# Autodesk Inventor assembly: SCLBRU5-35.0
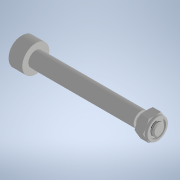
[picture p0: Inventor's stored thumbnail of the model, 180x180]
Saved by Autodesk Inventor 2021 (Build 250183000, 183)
## iProperties
Category: PARTsolutions
Company: MISUMI
Created: 2025-08-07
Part Number: SCLBRU5-35.0
Catalog Web Link: www.cadenas.de
Description: CLBR, CLBRH, PCLBR, PCLBRH, GCLBR, SCLBR, SCLBRH, GSCLBR, CLBRU, CLBRHU, PCLBRU, PCLBRHU, GCLBRU, SCLBRU, SCLBRHU, GSCLBRU-Hinge Pins - Lock Nut Type with Hexagon Socket Head
Vendor: MISUMI
Document SubType Name: Assembly
Designer: psAdmin
Manufacturer: MISUMI
Mass: 1.17278 g
Surface Area: 11.0588 cm^2
Volume: 1.17278 cm^3
Density: 1 g/cm^3
Title: SCLBRU5-35.0
Author: Cadenas PARTsolutions
Comments: Hinge Pins - Lock Nut Type with Hexagon Socket Head
PSOL_IDENT_0: {$CADENAS_DATA/23d-libs/misumi/metric/13_cantilever_shafts/clbr_asmtab.prj},343 {VTYP=3D},{STYP=ASST
PSOL_IDENT_1: AB},{NB=SCLBRU5-35.0},{LINA=SCLBRU5-35.0},{NN=CLBR, CLBRH, PCLBR, PCLBRH, GCLBR, SCLBR, SCLBRH, GSCL
PSOL_IDENT_2: BR, CLBRU, CLBRHU, PCLBRU, PCLBRHU, GCLBRU, SCLBRU, SCLBRHU, GSCLBRU},{DATE=21.04.2022 08:37:10},{GE
PSOL_IDENT_3: OMDATE=17.06.2021 12:28:52},{VERSION=},{LINEID=30},{WBVAR=MAT,HARD,ST,AC,L,ALT3,ALT2,MC,ALT1,FC,ALT4
PSOL_IDENT_4: },{WBNUMERIC=L,MC,FC}  {NB=SCLBRU5-35.0},{LINA=SCLBRU5-35.0},{KT=DUMMY},{PN=SCLBRU5-35.0},{TYPE=SCLB
PSOL_IDENT_5: RU},{MAT=SUS304},{HARD=1},{HARDALG= '1', '-' },{ST=},{STALG= '', '-' },{AC=UN},{ACALG= 'SN', 'Standa
PSOL_IDENT_6: rd Nuts', 'UN', 'U-Nuts' },{MATAC1=304 Stainless Steel (UNUTS)},{MATAC2=0},{STAC=0},{D=5},{L=35.0},{
PSOL_IDENT_7: L1=[10.0:100.0/0.1]},{LPN=35.0},{LPN1=35},{LPN2=0},{ALT3=},{A=9},{T=5},{ALT2=},{ALT2ALG= '' , 'Not a
PSOL_IDENT_8: pplicable' },{ALT2PN=},{MC=0},{MCALG=0},{M=M4},{M1=4},{M3D=4},{ALT1=},{ALT1ALG= '', 'w/o FC (Thread
PSOL_IDENT_9: Part Length)', '-FC', 'with FC (Thread Part Length)' },{ALT1PN=},{FC=0},{FCALG=0},{FCMIN1=4},{FCMAX1=
PSOL_IDENT_10: 5},{FCMIN2=7},{FCMAX2=12},{F=6},{F3D=6},{B=2.5},{E=2},{UU=4.9},{NN=1.5},{NUT=M4x0.7},{ALT4=},{HC=3.5
PSOL_IDENT_11: 0},{GG=1.2},{RR=0.3},{FF=3.1},{MAC=4},{BAC=7},{TAC=3.2},{CS=One side},{PPATH=clbr/clbr_templ.prj}
NB: SCLBRU5-35.0
NN: 1.5
NT: Hinge Pins - Lock Nut Type with Hexagon Socket Head
NBSYN: $PN.
LINA: SCLBRU5-35.0
CATALOG: Misumi
PN: SCLBRU5-35.0
MAT: SUS304
HARD: -
ST: -
AC: U-Nuts
D: 5
L: 35
ALT3: w/o LKC (L Dimension Tolerance)
A: 9
T: 5
ALT2: Not applicable
MC: 0
M: M4
ALT1: w/o FC (Thread Part Length)
FC: 0
F: 6
B: 2.5
E: 2
UU: 4.9
NUT: M4x0.7
ALT4: w/o HC (Shoulder Diameter Cut)
SUPPLIER: MISUMI
ARTICLENO: SCLBRU5-35.0
BOMINFO: SCLBRU5-35.0
CREATOR: CADENAS GmbH
## Documents named in this file (3)
- e:\temp\worker_COMMON_28\temp\tmp_5556_366_Hgir9\format_0\SCLBRU5-35_0.iam
- e:\temp\worker_COMMON_28\temp\tmp_5556_366_Hgir9\format_0\SCLBRU5-35_0_D.ipt
- e:\temp\worker_COMMON_28\temp\tmp_5556_366_Hgir9\format_0\UNUTZ4.ipt
## Components (2 placed, 2 different names)
1. SCLBRU5-35_0_D:1 — pin_to_nut_XY@1 <-> to_bolt_XY@2, pin_to_nut_Z@1 <-> to_bolt_Z@2, pin_to_nut_YZ@1 <-> to_bolt_YZ@2
2. UNUTZ4:1 — pin_to_nut_XY@1 <-> to_bolt_XY@2, pin_to_nut_Z@1 <-> to_bolt_Z@2, pin_to_nut_YZ@1 <-> to_bolt_YZ@2
## Relationships (3: Mate 2, Angle 1)
- pin_to_nut_XY@1 <-> to_bolt_XY@2 [Mate]: SCLBRU5-35_0_D:1 ↔ UNUTZ4:1
- pin_to_nut_Z@1 <-> to_bolt_Z@2 [Mate]: SCLBRU5-35_0_D:1 ↔ UNUTZ4:1
- pin_to_nut_YZ@1 <-> to_bolt_YZ@2 [Angle] (0 deg): SCLBRU5-35_0_D:1 ↔ UNUTZ4:1
